# Autodesk Inventor assembly: Body Chassis Assembly
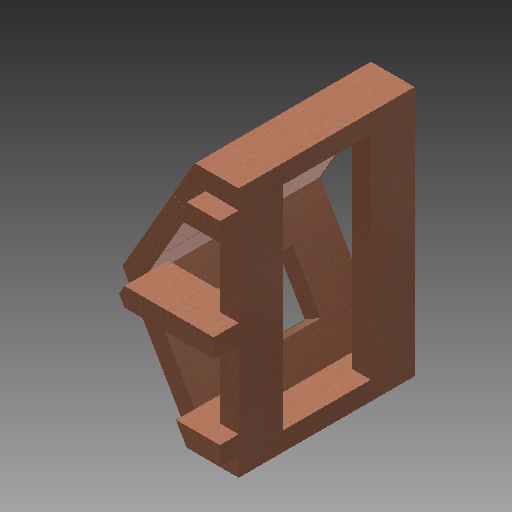
[picture p0: Inventor's stored thumbnail of the model, 512x512]
Saved by Autodesk Inventor 2017 (Build 210142000, 142)
## iProperties
Created: 2018-10-18
Part Number: Body Chassis Assembly
Document SubType Name: Assembly
Designer: Dell
Author: Dell
## Documents named in this file (7)
- C:\Users\Dell\Documents\GitHub\tr2\Body\Body Chassis Assembly.iam
- C:\Users\Dell\Documents\GitHub\tr2\Body\BO01.ipt
- C:\Users\Dell\Documents\GitHub\tr2\Body\BO02.ipt
- C:\Users\Dell\Documents\GitHub\tr2\Body\BO03.ipt
- C:\Users\Dell\Documents\GitHub\tr2\Body\BO04.ipt
- C:\Users\Dell\Documents\GitHub\tr2\Body\BO05.ipt
- C:\Users\Dell\Documents\GitHub\tr2\Body\BO06.ipt
## Components (15 placed, 6 different names)
1. BO01:1
2. BO01:2
3. BO02:1
4. BO02:2
5. BO01:3
6. BO01:4
7. BO02:3
8. BO02:4
9. BO01:5
10. BO01:6
11. BO03:1
12. BO03:2
13. BO04:1
14. BO05:1
15. BO06:1
## Relationships (42: Mate 23, Flush 19)
- [Mate]: BO01:1 ↔ BO01:2
- [Mate]: BO01:1 ↔ BO01:2
- [Flush]: BO01:1 ↔ BO01:2
- [Mate]: BO01:2 ↔ BO02:1
- [Flush]: BO01:2 ↔ BO02:1
- [Flush]: BO01:2 ↔ BO02:1
- [Mate]: BO01:2 ↔ BO02:2
- [Flush]: BO01:2 ↔ BO02:2
- [Flush]: BO01:2 ↔ BO02:2
- [Mate]: BO01:3 ↔ BO01:4
- [Mate]: BO01:3 ↔ BO01:4
- [Flush]: BO01:3 ↔ BO01:4
- [Mate]: BO01:4 ↔ BO02:3
- [Flush]: BO01:4 ↔ BO02:3
- [Flush]: BO01:4 ↔ BO02:3
- [Mate]: BO01:4 ↔ BO02:4
- [Flush]: BO01:4 ↔ BO02:4
- [Flush]: BO01:4 ↔ BO02:4
- [Mate]: BO02:1 ↔ BO01:3
- [Flush]: BO02:1 ↔ BO01:3
- [Flush]: BO02:1 ↔ BO01:3
- [Mate]: BO01:5 ↔ BO01:6
- [Mate]: BO01:5 ↔ BO01:6
- [Flush]: BO01:5 ↔ BO01:6
- [Mate]: BO02:3 ↔ BO01:5
- [Flush]: BO02:3 ↔ BO01:5
- [Flush]: BO02:3 ↔ BO01:5
- [Mate]: BO01:6 ↔ BO03:1
- [Flush]: BO01:6 ↔ BO03:1
- [Flush]: BO01:1 ↔ BO03:1
- [Flush]: BO01:1 ↔ BO03:2
- [Flush]: BO01:1 ↔ BO03:2
- [Mate]: BO01:1 ↔ BO03:2
- [Mate]: BO03:2 ↔ BO04:1
- [Mate]: BO03:2 ↔ BO04:1
- [Mate]: BO02:3 ↔ BO04:1
- [Mate]: BO01:2 ↔ BO05:1
- [Mate]: BO03:2 ↔ BO05:1
- [Mate]: BO03:2 ↔ BO05:1
- [Mate]: BO03:2 ↔ BO06:1
- [Mate]: BO03:2 ↔ BO06:1
- [Mate] (158.75 mm): BO04:1 ↔ BO06:1
## Named parameters: d0_d40 = 0 mm, d1_d41 = 0 mm, d8_d30 = 0 mm, d9_d31 = 0 mm, d10_d32 = 0 mm, d11_d33 = 0 mm, d12_d34 = 0 mm, d13_d35 = 0 mm, d14_d36 = 0 mm, d15_d37 = 0 mm, d16_d38 = 0 mm, d17_d39 = 0 mm, d12_d2 = 0 mm, d13_d3 = 0 mm, d14_d4 = 0 mm, d15_d5 = 0 mm, d16_d6 = 0 mm, d17_d7 = 0 mm, d18_d8 = 0 mm, d19_d0 = 0 mm, d20_d1 = 0 mm, d24_d2 = 0 mm, d28_d0 = 0 mm, d29_d1 = 0 mm
